# Autodesk Inventor assembly: A_Fuselage
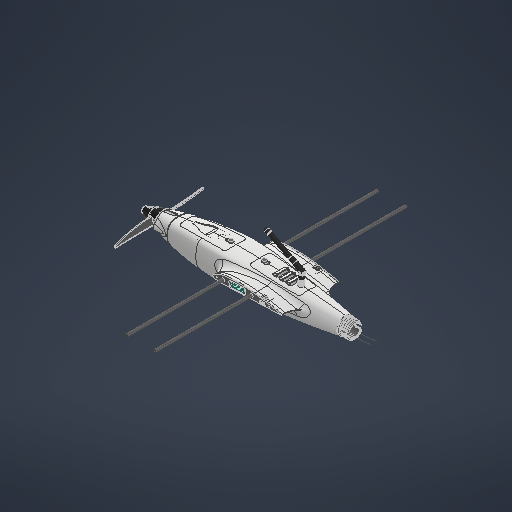
[picture p0: Inventor's stored thumbnail of the model, 512x512]
Saved by Autodesk Inventor 2026 (Build 300175000, 175)
## iProperties
Created: 2025-09-10
Part Number: A_Fuselage
Document SubType Name: Assembly
Designer: FAL
Author: FAL
## iProperties of the stored document MemberDocs/xRgsxtxc0Ms1ywvfrKsg1cec31d
Created: 2025-09-10
Part Number: A_Fuselage
Document SubType Name: Assembly
Designer: FAL
Author: FAL
## iProperties of the stored document MemberDocs/xF1najkv1Jkw2aegrIkppqzyyJd
Created: 2025-09-10
Part Number: A_Fuselage
Document SubType Name: Assembly
Designer: FAL
Author: FAL
## Documents named in this file (28)
- C:\Users\FAL\Projekte\Git\AIRBERT\CAD\Fuselage\A_Fuselage.iam
- C:\Users\FAL\Projekte\Git\AIRBERT\CAD\Fuselage\P_fuselage_body_back.ipt
- C:\Users\FAL\Projekte\Git\AIRBERT\CAD\Fuselage\P_Fuselage_body_front.ipt
- C:\Users\FAL\Projekte\Git\AIRBERT\CAD\Fuselage\P_Fuselage_Body_groundplate.ipt
- C:\Users\FAL\Projekte\Git\AIRBERT\CAD\Fuselage\P_fuselage_body_mid.ipt
- C:\Users\FAL\Projekte\Git\AIRBERT\CAD\Fuselage\P_Fuselage_body_pipe_connector_inlet.ipt
- C:\Users\FAL\Projekte\Git\AIRBERT\CAD\Fuselage\P_Fuselage_body_pipe_connector_nut.ipt
- C:\Users\FAL\Projekte\Git\AIRBERT\CAD\Fuselage\P_Fuselage_cap_front.ipt
- C:\Users\FAL\Projekte\Git\AIRBERT\CAD\Fuselage\P_Fuselage_cap_mid.ipt
- C:\Users\FAL\Projekte\Git\AIRBERT\CAD\Fuselage\P_Fuselage_Nose.ipt
- C:\Users\FAL\Projekte\Git\AIRBERT\CAD\Fuselage\P_MotorBackplate.ipt
- C:\Users\FAL\Projekte\Git\AIRBERT\CAD\Fuselage\P_MotorNose.ipt
- C:\Users\FAL\Projekte\Git\AIRBERT\CAD\Fuselage\P_Carbonpipe_6mm.ipt
- C:\Users\FAL\Projekte\Git\AIRBERT\CAD\Fuselage\openmechanism\A_openmechanism.iam
- C:\Users\FAL\Projekte\Git\AIRBERT\CAD\Fuselage\P_Fuselage_Wingplate.ipt
- C:\Users\FAL\Projekte\Git\AIRBERT\CAD\Electronic\P_ESC_40A.ipt
- C:\Users\FAL\Projekte\Git\AIRBERT\CAD\Electronic\P_Receiver_Radiolink.ipt
- C:\Users\FAL\Projekte\Git\AIRBERT\CAD\Electronic\P_Akku_Dummy.ipt
- C:\Users\FAL\Projekte\Git\AIRBERT\CAD\Electronic\P_BLDC_2200KV.ipt
- C:\Users\FAL\Projekte\Git\AIRBERT\CAD\Electronic\Flightcontroller_PCB\A_Flightcontroller_PCB.iam
- C:\Users\FAL\Projekte\Git\AIRBERT\CAD\Electronic\P_JX9_M_ref.ipt
- C:\Users\FAL\Projekte\Git\AIRBERT\CAD\Fuselage\P_Fuselage_Body.ipt
- C:\Users\FAL\Projekte\Git\AIRBERT\CAD\Fuselage\P_Fuselage_PinButton.ipt
- C:\Users\FAL\Projekte\Git\AIRBERT\CAD\Electronic\Antenna\Antenna_Dfaut.iam
- C:\Users\FAL\Projekte\Git\AIRBERT\CAD\Fuselage\mirror\P_Fuselage_Wingplate_MIR.ipt
- C:\Users\FAL\Projekte\Git\AIRBERT\CAD\Fuselage\mirror\P_Fuselage_PinButton_MIR.ipt
- C:\Users\FAL\Projekte\Git\AIRBERT\CAD\Fuselage\mirror\P_JX9_M_ref_MIR.ipt
- C:\Users\FAL\Projekte\Git\AIRBERT\CAD\Fuselage\P_Fuselage_prop.ipt
## Components (29 placed, 27 different names)
1. P_fuselage_body_back:1 — Fluchtend:4, Fluchtend:5, Fluchtend:6
2. P_Fuselage_body_front:1 — Fluchtend:7, Fluchtend:8, Fluchtend:9, Passend:15
3. P_Fuselage_Body_groundplate:1 — Fluchtend:10, Fluchtend:11, Fluchtend:12, Passend:16, Passend:17, Passend:18, Passend:19, Passend:20, Passend:21
4. P_fuselage_body_mid:1 — Fluchtend:13, Fluchtend:14, Fluchtend:15, Passend:22
5. P_Fuselage_body_pipe_connector_inlet:1 — Fluchtend:16, Fluchtend:17, Fluchtend:18
6. P_Fuselage_body_pipe_connector_nut:1 — Fluchtend:19, Fluchtend:20, Fluchtend:21
7. P_Fuselage_cap_front:1 — Fluchtend:22, Fluchtend:23, Fluchtend:24, Passend:35, Passend:36
8. P_Fuselage_cap_mid:1 — Fluchtend:25, Fluchtend:26, Fluchtend:27, Passend:23, Passend:24, Passend:63, Passend:64
9. P_Fuselage_Nose:1 — Fluchtend:28, Fluchtend:29, Fluchtend:30, Passend:34
10. P_MotorBackplate:1 — Fluchtend:31, Fluchtend:32, Fluchtend:33, Passend:32, Passend:33
11. P_MotorNose:1 — Fluchtend:34, Fluchtend:35, Fluchtend:36
12. P_Carbonpipe_6mm:1 — Fluchtend:37
13. P_Carbonpipe_6mm:2 — Fluchtend:38
14. A_openmechanism:1 [sub-assembly] — Passend:62, Passend:63, Passend:64
15. A_openmechanism:2 [sub-assembly] — Passend:35, Fluchtend:60, Passend:36
16. P_Fuselage_Wingplate:1 — Fluchtend:42, Fluchtend:43, Fluchtend:44
17. P_Fuselage_PinButton:1 — Fluchtend:55, Fluchtend:56, Fluchtend:57
18. P_Fuselage_prop:1 — Passend:29, Passend:30, Passend:34
19. Antenna_Dfaut:1 [sub-assembly] — Passend:23, Passend:24
20. P_JX9_M_ref:1 — Passend:22
21. P_ESC_40A:1
22. P_Receiver_Radiolink:1 — Passend:16, Passend:21
23. P_Akku_Dummy:1 — Fluchtend:45, Passend:15, Passend:17, Passend:20
24. P_BLDC_2200KV:1 — Passend:11, Passend:29, Passend:32, Passend:33
25. A_Flightcontroller_PCB:1 [sub-assembly] — Passend:13, Passend:18, Passend:19
26. P_Fuselage_Wingplate_MIR:1 — Passend:26, Fluchtend:58
27. P_Fuselage_PinButton_MIR:1 — Passend:28, Fluchtend:59
28. P_JX9_M_ref_MIR:1
29. P_Fuselage_Body:1 — Fluchtend:52, Fluchtend:53, Fluchtend:54
## Relationships (72: Flush 48, Mate 24)
- Fluchtend:4 [Flush]: P_fuselage_body_back:1
- Fluchtend:5 [Flush]: P_fuselage_body_back:1
- Fluchtend:6 [Flush]: P_fuselage_body_back:1
- Fluchtend:7 [Flush]: P_Fuselage_body_front:1
- Fluchtend:8 [Flush]: P_Fuselage_body_front:1
- Fluchtend:9 [Flush]: P_Fuselage_body_front:1
- Fluchtend:10 [Flush]: P_Fuselage_Body_groundplate:1
- Fluchtend:11 [Flush]: P_Fuselage_Body_groundplate:1
- Fluchtend:12 [Flush]: P_Fuselage_Body_groundplate:1
- Fluchtend:13 [Flush]: P_fuselage_body_mid:1
- Fluchtend:14 [Flush]: P_fuselage_body_mid:1
- Fluchtend:15 [Flush]: P_fuselage_body_mid:1
- Fluchtend:16 [Flush]: P_Fuselage_body_pipe_connector_inlet:1
- Fluchtend:17 [Flush]: P_Fuselage_body_pipe_connector_inlet:1
- Fluchtend:18 [Flush]: P_Fuselage_body_pipe_connector_inlet:1
- Fluchtend:19 [Flush]: P_Fuselage_body_pipe_connector_nut:1
- Fluchtend:20 [Flush]: P_Fuselage_body_pipe_connector_nut:1
- Fluchtend:21 [Flush]: P_Fuselage_body_pipe_connector_nut:1
- Fluchtend:22 [Flush]: P_Fuselage_cap_front:1
- Fluchtend:23 [Flush]: P_Fuselage_cap_front:1
- Fluchtend:24 [Flush]: P_Fuselage_cap_front:1
- Fluchtend:25 [Flush]: P_Fuselage_cap_mid:1
- Fluchtend:26 [Flush]: P_Fuselage_cap_mid:1
- Fluchtend:27 [Flush]: P_Fuselage_cap_mid:1
- Fluchtend:28 [Flush]: P_Fuselage_Nose:1
- Fluchtend:29 [Flush]: P_Fuselage_Nose:1
- Fluchtend:30 [Flush]: P_Fuselage_Nose:1
- Fluchtend:31 [Flush]: P_MotorBackplate:1
- Fluchtend:32 [Flush]: P_MotorBackplate:1
- Fluchtend:33 [Flush]: P_MotorBackplate:1
- Fluchtend:34 [Flush] (2 mm): P_MotorNose:1
- Fluchtend:35 [Flush]: P_MotorNose:1
- Fluchtend:36 [Flush]: P_MotorNose:1
- Fluchtend:37 [Flush]: P_Carbonpipe_6mm:1
- Fluchtend:38 [Flush]: P_Carbonpipe_6mm:2
- Fluchtend:42 [Flush]: P_Fuselage_Wingplate:1
- Fluchtend:43 [Flush]: P_Fuselage_Wingplate:1
- Fluchtend:44 [Flush]: P_Fuselage_Wingplate:1
- Passend:11 [Mate]: P_BLDC_2200KV:1
- Fluchtend:45 [Flush]: P_Akku_Dummy:1
- Passend:13 [Mate]: A_Flightcontroller_PCB:1
- Fluchtend:52 [Flush]: P_Fuselage_Body:1
- Fluchtend:53 [Flush]: P_Fuselage_Body:1
- Fluchtend:54 [Flush]: P_Fuselage_Body:1
- Passend:15 [Mate]: P_Fuselage_body_front:1 ↔ P_Akku_Dummy:1
- Passend:16 [Mate]: P_Fuselage_Body_groundplate:1 ↔ P_Receiver_Radiolink:1
- Passend:17 [Mate]: P_Fuselage_Body_groundplate:1 ↔ P_Akku_Dummy:1
- Passend:18 [Mate]: P_Fuselage_Body_groundplate:1 ↔ A_Flightcontroller_PCB:1
- Passend:19 [Mate]: P_Fuselage_Body_groundplate:1 ↔ A_Flightcontroller_PCB:1
- Passend:20 [Mate]: P_Fuselage_Body_groundplate:1 ↔ P_Akku_Dummy:1
- Passend:21 [Mate]: P_Fuselage_Body_groundplate:1 ↔ P_Receiver_Radiolink:1
- Passend:22 [Mate]: P_fuselage_body_mid:1 ↔ P_JX9_M_ref:1
- Fluchtend:55 [Flush]: P_Fuselage_PinButton:1
- Fluchtend:56 [Flush]: P_Fuselage_PinButton:1
- Fluchtend:57 [Flush]: P_Fuselage_PinButton:1
- Passend:23 [Mate]: P_Fuselage_cap_mid:1 ↔ Antenna_Dfaut:1
- Passend:24 [Mate]: P_Fuselage_cap_mid:1 ↔ Antenna_Dfaut:1
- Passend:26 [Mate]: P_Fuselage_Wingplate_MIR:1
- Fluchtend:58 [Flush]: P_Fuselage_Wingplate_MIR:1
- Passend:28 [Mate]: P_Fuselage_PinButton_MIR:1
- Fluchtend:59 [Flush]: P_Fuselage_PinButton_MIR:1
- Passend:29 [Mate]: P_Fuselage_prop:1 ↔ P_BLDC_2200KV:1
- Passend:30 [Mate]: P_Fuselage_prop:1
- Passend:32 [Mate]: P_MotorBackplate:1 ↔ P_BLDC_2200KV:1
- Passend:33 [Mate]: P_MotorBackplate:1 ↔ P_BLDC_2200KV:1
- Passend:34 [Mate] (6 mm): P_Fuselage_Nose:1 ↔ P_Fuselage_prop:1
- Passend:35 [Mate]: P_Fuselage_cap_front:1 ↔ A_openmechanism:2
- Fluchtend:60 [Flush]: A_openmechanism:2
- Passend:36 [Mate] (0.25 mm): P_Fuselage_cap_front:1 ↔ A_openmechanism:2
- Passend:62 [Mate]: A_openmechanism:1
- Passend:63 [Mate] (0.25 mm): P_Fuselage_cap_mid:1 ↔ A_openmechanism:1
- Passend:64 [Mate] (3 mm): P_Fuselage_cap_mid:1 ↔ A_openmechanism:1
